# Autodesk Inventor assembly: Flex Assembly
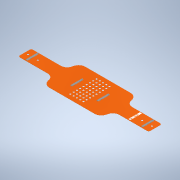
[picture p0: Inventor's stored thumbnail of the model, 180x180]
Saved by Autodesk Inventor 2022 (Build 260153000, 153)
## iProperties
Created: 2021-07-16
Part Number: Flex Assembly
Document SubType Name: Assembly
Designer: Caleb
Author: Caleb
## Documents named in this file (3)
- C:\Users\Caleb\Desktop\nebraska-silicon-lab\Hardware\ETL\Module Assembly\Tamale Assembly Plate\Flex Assembly.iam
- C:\Users\Caleb\Desktop\nebraska-silicon-lab\Hardware\ETL\Module Assembly\Tamale Assembly Plate\Flex.ipt
- C:\Users\Caleb\Desktop\nebraska-silicon-lab\Hardware\ETL\Module Assembly\Tamale Assembly Plate\Board to board, F.ipt
## Components (5 placed, 2 different names)
1. Flex:1 — Mate:1, Mate:2, Mate:3, Mate:4, Angle:1, Angle:2, Angle:3, Angle:4, Flush:1, Flush:2, Flush:6, Flush:7, Flush:8
2. Board to board, F:1 — Mate:1, Angle:4, Flush:2, Flush:3, Flush:6
3. Board to board, F:2 — Mate:2, Angle:3, Flush:3, Flush:4, Flush:7
4. Board to board, F:3 — Mate:3, Angle:2, Flush:4, Flush:5, Flush:8
5. Board to board, F:4 — Mate:4, Angle:1, Flush:1, Flush:5
## Relationships (16: Flush 8, Mate 4, Angle 4)
- Mate:1: Flex:1 ↔ Board to board, F:1
- Mate:2: Flex:1 ↔ Board to board, F:2
- Mate:3: Flex:1 ↔ Board to board, F:3
- Mate:4: Flex:1 ↔ Board to board, F:4
- Angle:1 (0 deg): Flex:1 ↔ Board to board, F:4
- Angle:2 (0 deg): Flex:1 ↔ Board to board, F:3
- Angle:3 (0 deg): Flex:1 ↔ Board to board, F:2
- Angle:4 (0 deg): Flex:1 ↔ Board to board, F:1
- Flush:1 (6.6675 mm): Flex:1 ↔ Board to board, F:4
- Flush:2 (6.6675 mm): Flex:1 ↔ Board to board, F:1
- Flush:3: Board to board, F:1 ↔ Board to board, F:2
- Flush:4: Board to board, F:2 ↔ Board to board, F:3
- Flush:5: Board to board, F:3 ↔ Board to board, F:4
- Flush:6 (0.6477 mm): Flex:1 ↔ Board to board, F:1
- Flush:7 (50.0888 mm): Flex:1 ↔ Board to board, F:2
- Flush:8 (50.0888 mm): Flex:1 ↔ Board to board, F:3
